# Autodesk Inventor assembly: rovPrototype1
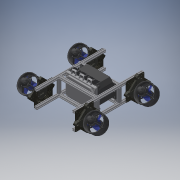
[picture p0: Inventor's stored thumbnail of the model, 180x180]
Saved by Autodesk Inventor 2018 (Build 220112000, 112)
## iProperties
Created: 2019-02-03
Part Number: rovPrototype1
Document SubType Name: Assembly
Designer: anirudh
Author: anirudh
## Documents named in this file (8)
- C:\Users\anirudh\Documents\MARS Fund\MATE Robotics\Silicon Sharks\2018-2019\Prototype1\rovPrototype1.iam
- C:\Users\anirudh\Documents\MARS Fund\MATE Robotics\Silicon Sharks\2018-2019\Prototype1\15inREV.ipt
- C:\Users\anirudh\Documents\MARS Fund\MATE Robotics\Silicon Sharks\2018-2019\Prototype1\12inREV.ipt
- C:\Users\anirudh\Documents\MARS Fund\MATE Robotics\Silicon Sharks\2018-2019\Prototype1\4inREV.ipt
- C:\Users\anirudh\Documents\MARS Fund\MATE Robotics\Silicon Sharks\2018-2019\Prototype1\LazySusanBearing.ipt
- C:\Users\anirudh\Documents\MARS Fund\MATE Robotics\Silicon Sharks\2018-2019\Prototype1\ThrusterMount.ipt
- C:\Users\anirudh\Documents\MARS Fund\MATE Robotics\Silicon Sharks\2018-2019\Prototype1\T200-THRUSTER-R1.ipt
- C:\Users\anirudh\Documents\MARS Fund\MATE Robotics\Silicon Sharks\2018-2019\Electrical Housing\DaSmallerBox.iam
## Components (27 placed, 7 different names)
1. 15inREV:1 — Flush:3, Flush:4, Mate:2, Flush:5, Flush:6, Mate:3, Mate:5, Mate:6, Flush:12, Flush:19, Flush:21, Symmetry:1, Mate:51, Flush:71, Flush:72, Mate:52, Flush:73, Flush:74, Flush:79
2. 15inREV:2 — Flush:3, Flush:4, Mate:2, Flush:14, Mate:10, Mate:11
3. 15inREV:3 — Flush:1, Flush:2, Mate:1, Flush:5, Flush:6, Mate:3, Mate:4, Flush:7, Flush:11, Mate:7, Flush:15, Flush:17, Symmetry:1, Mate:55, Flush:80, Flush:81, Mate:56, Flush:82, Flush:83
4. 15inREV:4 — Flush:1, Flush:2, Mate:1, Flush:10, Mate:8, Mate:9
5. 12inREV:1 — Flush:13, Mate:7, Flush:14, Flush:66, Mate:44
6. 12inREV:2 — Flush:11, Mate:6, Flush:12, Flush:13, Flush:18, Flush:22, Mate:42, Flush:65, Mate:71, Flush:88
7. 12inREV:3 — Flush:9, Mate:5, Flush:10
8. 12inREV:4 — Mate:4, Flush:7, Flush:9, Flush:16, Flush:20, Flush:79
9. 4inREV:1 — Flush:15, Flush:16, Mate:8
10. 4inREV:2 — Flush:21, Flush:22, Mate:11, Mate:43, Flush:89
11. 4inREV:3 — Flush:17, Flush:18, Mate:9, Mate:45
12. 4inREV:4 — Flush:19, Flush:20, Mate:10
13. 4inREV:5 — Mate:42, Mate:43, Flush:65
14. 4inREV:6 — Flush:66, Mate:44, Mate:45
15. LazySusanBearing:1 — Mate:51, Flush:71, Flush:72, Mate:53, Flush:75, Flush:76
16. LazySusanBearing:2 — Mate:52, Flush:73, Flush:74, Mate:54, Flush:77, Flush:78
17. ThrusterMount:1 — Mate:53, Flush:75, Flush:76, Mate:59, Mate:60, Mate:61
18. ThrusterMount:2 — Mate:54, Flush:77, Flush:78, Mate:62, Mate:63, Mate:64
19. LazySusanBearing:3 — Mate:55, Flush:80, Flush:81, Mate:57, Flush:84, Flush:86
20. LazySusanBearing:4 — Mate:56, Flush:82, Flush:83, Mate:58, Flush:85, Flush:87
21. ThrusterMount:3 — Mate:57, Flush:85, Flush:87, Mate:66, Mate:67, Mate:68
22. ThrusterMount:4 — Mate:58, Flush:84, Flush:86, Mate:65, Mate:69, Mate:70
23. T200-THRUSTER-R1:1 — Mate:59, Mate:60, Mate:61
24. T200-THRUSTER-R1:2 — Mate:62, Mate:63, Mate:64
25. T200-THRUSTER-R1:3 — Mate:65, Mate:69, Mate:70
26. T200-THRUSTER-R1:4 — Mate:66, Mate:67, Mate:68
27. DaSmallerBox:1 [sub-assembly] — Mate:71, Flush:88, Flush:89
## Relationships (79: Flush 42, Mate 36, Symmetry 1)
- Flush:1: 15inREV:3 ↔ 15inREV:4
- Flush:2: 15inREV:3 ↔ 15inREV:4
- Mate:1 (71.6 mm): 15inREV:3 ↔ 15inREV:4
- Flush:3: 15inREV:1 ↔ 15inREV:2
- Flush:4: 15inREV:1 ↔ 15inREV:2
- Mate:2 (71.6 mm): 15inREV:1 ↔ 15inREV:2
- Flush:5: 15inREV:1 ↔ 15inREV:3
- Flush:6: 15inREV:1 ↔ 15inREV:3
- Mate:3 (195.263 mm): 15inREV:1 ↔ 15inREV:3
- Mate:4: 15inREV:3 ↔ 12inREV:4
- Flush:7: 15inREV:3 ↔ 12inREV:4
- Flush:9: 12inREV:3 ↔ 12inREV:4
- Mate:5: 15inREV:1 ↔ 12inREV:3
- Flush:10: 15inREV:4 ↔ 12inREV:3
- Flush:11: 15inREV:3 ↔ 12inREV:2
- Mate:6: 15inREV:1 ↔ 12inREV:2
- Flush:12 (-121.5898 mm): 15inREV:1 ↔ 12inREV:2
- Flush:13: 12inREV:1 ↔ 12inREV:2
- Mate:7: 15inREV:3 ↔ 12inREV:1
- Flush:14: 15inREV:2 ↔ 12inREV:1
- Flush:15: 15inREV:3 ↔ 4inREV:1
- Flush:16: 12inREV:4 ↔ 4inREV:1
- Mate:8: 15inREV:4 ↔ 4inREV:1
- Flush:17: 15inREV:3 ↔ 4inREV:3
- Flush:18: 12inREV:2 ↔ 4inREV:3
- Mate:9: 15inREV:4 ↔ 4inREV:3
- Flush:19: 15inREV:1 ↔ 4inREV:4
- Flush:20: 12inREV:4 ↔ 4inREV:4
- Mate:10: 15inREV:2 ↔ 4inREV:4
- Flush:21: 15inREV:1 ↔ 4inREV:2
- Flush:22: 12inREV:2 ↔ 4inREV:2
- Mate:11: 15inREV:2 ↔ 4inREV:2
- Symmetry:1: 15inREV:1 ↔ 15inREV:3
- Mate:42: 12inREV:2 ↔ 4inREV:5
- Mate:43: 4inREV:2 ↔ 4inREV:5
- Flush:65: 12inREV:2 ↔ 4inREV:5
- Flush:66: 12inREV:1 ↔ 4inREV:6
- Mate:44: 12inREV:1 ↔ 4inREV:6
- Mate:45: 4inREV:3 ↔ 4inREV:6
- Mate:51: 15inREV:1 ↔ LazySusanBearing:1
- Flush:71: 15inREV:1 ↔ LazySusanBearing:1
- Flush:72: 15inREV:1 ↔ LazySusanBearing:1
- Mate:52: 15inREV:1 ↔ LazySusanBearing:2
- Flush:73: 15inREV:1 ↔ LazySusanBearing:2
- Flush:74: 15inREV:1 ↔ LazySusanBearing:2
- Mate:53: LazySusanBearing:1 ↔ ThrusterMount:1
- Flush:75 (10.3124 mm): LazySusanBearing:1 ↔ ThrusterMount:1
- Flush:76 (10.3124 mm): LazySusanBearing:1 ↔ ThrusterMount:1
- Mate:54: LazySusanBearing:2 ↔ ThrusterMount:2
- Flush:77 (10.3124 mm): LazySusanBearing:2 ↔ ThrusterMount:2
- Flush:78 (10.3124 mm): LazySusanBearing:2 ↔ ThrusterMount:2
- Flush:79 (121.5898 mm): 15inREV:1 ↔ 12inREV:4
- Mate:55: 15inREV:3 ↔ LazySusanBearing:3
- Flush:80: 15inREV:3 ↔ LazySusanBearing:3
- Flush:81: 15inREV:3 ↔ LazySusanBearing:3
- Mate:56: 15inREV:3 ↔ LazySusanBearing:4
- Flush:82: 15inREV:3 ↔ LazySusanBearing:4
- Flush:83: 15inREV:3 ↔ LazySusanBearing:4
- Mate:57: LazySusanBearing:3 ↔ ThrusterMount:3
- Mate:58: LazySusanBearing:4 ↔ ThrusterMount:4
- Flush:84 (10.3124 mm): LazySusanBearing:3 ↔ ThrusterMount:4
- Flush:85 (10.3124 mm): LazySusanBearing:4 ↔ ThrusterMount:3
- Flush:86 (10.3124 mm): LazySusanBearing:3 ↔ ThrusterMount:4
- Flush:87 (10.3124 mm): LazySusanBearing:4 ↔ ThrusterMount:3
- Mate:59: ThrusterMount:1 ↔ T200-THRUSTER-R1:1
- Mate:60: ThrusterMount:1 ↔ T200-THRUSTER-R1:1
- Mate:61: ThrusterMount:1 ↔ T200-THRUSTER-R1:1
- Mate:62: ThrusterMount:2 ↔ T200-THRUSTER-R1:2
- Mate:63: ThrusterMount:2 ↔ T200-THRUSTER-R1:2
- Mate:64: ThrusterMount:2 ↔ T200-THRUSTER-R1:2
- Mate:65: ThrusterMount:4 ↔ T200-THRUSTER-R1:3
- Mate:66: ThrusterMount:3 ↔ T200-THRUSTER-R1:4
- Mate:67: ThrusterMount:3 ↔ T200-THRUSTER-R1:4
- Mate:68: ThrusterMount:3 ↔ T200-THRUSTER-R1:4
- Mate:69: ThrusterMount:4 ↔ T200-THRUSTER-R1:3
- Mate:70: ThrusterMount:4 ↔ T200-THRUSTER-R1:3
- Mate:71: 12inREV:2 ↔ DaSmallerBox:1
- Flush:88: 12inREV:2 ↔ DaSmallerBox:1
- Flush:89 (15 mm): 4inREV:2 ↔ DaSmallerBox:1
